# Autodesk Inventor assembly: Full_model
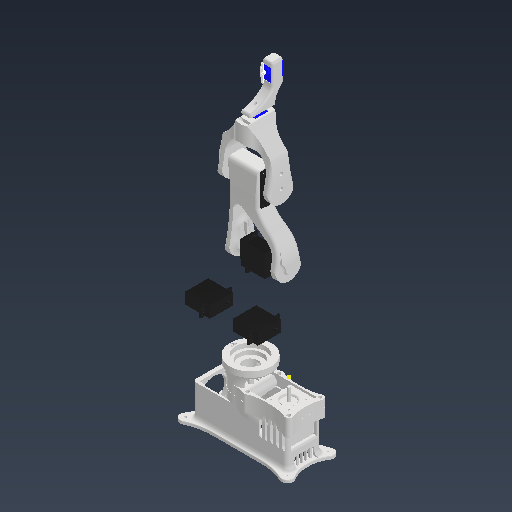
[picture p0: Inventor's stored thumbnail of the model, 512x512]
Saved by Autodesk Inventor 2026.1 (Build 301233020, 233B)
## iProperties
Created: 2025-08-29
Part Number: Full_model
Document SubType Name: Assembly
Designer: Piter
Author: Piter
## Documents named in this file (12)
- C:\Users\Piter\OneDrive\Pulpit\Robots\david_Arm\Davie-Robot-Arm\3D Models\Full_model.iam
- C:\Users\Piter\OneDrive\Pulpit\Robots\david_Arm\Davie-Robot-Arm\3D Models\Arm2.ipt
- C:\Users\Piter\OneDrive\Pulpit\Robots\david_Arm\Davie-Robot-Arm\3D Models\Component models\feetech_25kg_servo.ipt
- C:\Users\Piter\OneDrive\Pulpit\Robots\david_Arm\Davie-Robot-Arm\3D Models\Arm3.ipt
- C:\Users\Piter\OneDrive\Pulpit\Robots\david_Arm\Davie-Robot-Arm\3D Models\Component models\TowerPro SG90 M.ipt
- C:\Users\Piter\OneDrive\Pulpit\Robots\david_Arm\Davie-Robot-Arm\3D Models\Arm4.ipt
- C:\Users\Piter\OneDrive\Pulpit\Robots\david_Arm\Davie-Robot-Arm\3D Models\Arm1_2servos.ipt
- C:\Users\Piter\OneDrive\Pulpit\Robots\david_Arm\Davie-Robot-Arm\3D Models\Axis1_v2.ipt
- C:\Users\Piter\OneDrive\Pulpit\Robots\david_Arm\Davie-Robot-Arm\3D Models\Base_top.ipt
- C:\Users\Piter\OneDrive\Pulpit\Robots\david_Arm\Davie-Robot-Arm\3D Models\Base_bottom.ipt
- C:\Users\Piter\OneDrive\Pulpit\Robots\david_Arm\Davie-Robot-Arm\3D Models\Component models\Slip_ring.ipt
- C:\Users\Piter\OneDrive\Pulpit\Robots\david_Arm\Davie-Robot-Arm\3D Models\Component models\Stepper.ipt
## Components (15 placed, 11 different names)
1. Arm2:1 — Rotational:4, Rotational:6, Rigid:7
2. feetech_25kg_servo:1 — Rigid:6
3. Arm3:1 — Rotational:4, Rigid:1
4. TowerPro SG90 M:1 — Rigid:1, Rotational:5
5. Arm4:1 — Rotational:5, Rigid:5
6. TowerPro SG90 M:2 — Rigid:5
7. Arm1_2servos:1 — Rigid:6, Rotational:6, Rotational:8
8. feetech_25kg_servo:2 — Rigid:7
9. feetech_25kg_servo:3 — Rigid:9
10. feetech_25kg_servo:4 — Rigid:8
11. Axis1_v2:1 — Rigid:8, Rigid:9, Rotational:8, Rotational:10
12. Base_top:1 — Rotational:10, Rigid:10, Rigid:11, Rigid:12
13. Base_bottom:1 — Rigid:10, Mate:1
14. Slip_ring:1 — Rigid:11, Mate:2
15. Stepper:1 — Rigid:12
## Relationships (17: WeldJoint 9, RevoluteJoint 5, Mate 3)
- Rotational:4 [RevoluteJoint]: Arm2:1 ↔ Arm3:1
- Rigid:1 [WeldJoint]: Arm3:1 ↔ TowerPro SG90 M:1
- Rotational:5 [RevoluteJoint]: TowerPro SG90 M:1 ↔ Arm4:1
- Rigid:5 [WeldJoint]: Arm4:1 ↔ TowerPro SG90 M:2
- Rigid:6 [WeldJoint]: feetech_25kg_servo:1 ↔ Arm1_2servos:1
- Rotational:6 [RevoluteJoint]: Arm2:1 ↔ Arm1_2servos:1
- Rigid:7 [WeldJoint]: Arm2:1 ↔ feetech_25kg_servo:2
- Rigid:8 [WeldJoint]: feetech_25kg_servo:4 ↔ Axis1_v2:1
- Rigid:9 [WeldJoint]: feetech_25kg_servo:3 ↔ Axis1_v2:1
- Rotational:8 [RevoluteJoint]: Arm1_2servos:1 ↔ Axis1_v2:1
- Rotational:10 [RevoluteJoint] (-1 mm): Axis1_v2:1 ↔ Base_top:1
- Rigid:10 [WeldJoint]: Base_top:1 ↔ Base_bottom:1
- Rigid:11 [WeldJoint]: Base_top:1 ↔ Slip_ring:1
- Rigid:12 [WeldJoint]: Base_top:1 ↔ Stepper:1
- Mate:1: Base_bottom:1
- Mate:2: Slip_ring:1
- Mate:3
